# Autodesk Inventor assembly: 18-025-003
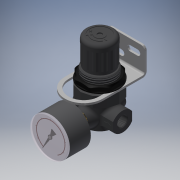
[picture p0: Inventor's stored thumbnail of the model, 180x180]
Saved by Autodesk Inventor 2017.1 (Build 211199000, 199)
## iProperties
Category: Bag  #9
Company: Autodesk Inc.
Created: 2016-12-23
Part Number: 18-025-003
Document SubType Name: Assembly
Designer: Autodesk Inc.
Catalog Web Link: http://www.norgren.com/document_resources/EN/8.300.200.PDF
Vendor: Norgren
Description: Main Regulator (assembled)
Author: Autodesk Inc.
Keywords: Yellow Tote
## Documents named in this file (5)
- D:\FIRST\FIRST KOP 2017\FIRST 2017 Yellow Tote\18-025-003.iam
- D:\FIRST\FIRST KOP 2017\FIRST 2017 Yellow Tote\R07-100-RNEA.ipt
- D:\FIRST\FIRST KOP 2017\FIRST 2017 Yellow Tote\Parts\Pneumatics_Norgren_18-025-003_Bracket.ipt
- D:\FIRST\FIRST KOP 2017\FIRST 2017 Yellow Tote\Parts\Pneumatics_Norgren_18-025-003_Panel Nut.ipt
- D:\FIRST\FIRST KOP 2017\FIRST 2017 Yellow Tote\18-013-212.iam
## Components (4 placed, 4 different names)
1. R07-100-RNEA:1 — Mate:1, Mate:2, Mate:3, Insert:1
2. Pneumatics_Norgren_18-025-003_Bracket:1 — Mate:1, Mate:2, Mate:4
3. Pneumatics_Norgren_18-025-003_Panel Nut:1 — Mate:3, Mate:4
4. 18-013-212:1 [sub-assembly] — Insert:1
## Relationships (5: Mate 4, Insert 1)
- Mate:1: R07-100-RNEA:1 ↔ Pneumatics_Norgren_18-025-003_Bracket:1
- Mate:2: R07-100-RNEA:1 ↔ Pneumatics_Norgren_18-025-003_Bracket:1
- Mate:3: R07-100-RNEA:1 ↔ Pneumatics_Norgren_18-025-003_Panel Nut:1
- Mate:4: Pneumatics_Norgren_18-025-003_Bracket:1 ↔ Pneumatics_Norgren_18-025-003_Panel Nut:1
- Insert:1: R07-100-RNEA:1 ↔ 18-013-212:1
